# Autodesk Inventor assembly: EFOI-10
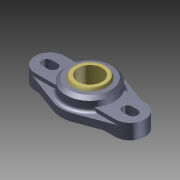
[picture p0: Inventor's stored thumbnail of the model, 180x180]
Saved by Autodesk Inventor 2011 (Build 150239000, 239)
## iProperties
Category: Plastic Bearings
Created: 2007-11-11
Part Number: EFOI-10
Catalog Web Link: http://www.igus.com/igcat/ig_cat1.asp?p=ig_27_2.gif
Description: igubal Flange Bearing
Vendor: igus
Document SubType Name: Assembly
Mass: 17.3933 g
Surface Area: 82.1485 cm^2
Volume: 15.021 cm^3
Density: 1.15793 g/cm^3
Project: FIRST
Title: igubal Flange Bearing
Author: Autodesk, Inc.
## Documents named in this file (3)
- R:\2012\Inventor\vkop\Plastic-Bearings\Plastic Bearings_igus_EFOI-10.iam
- R:\2012\Inventor\vkop\Plastic-Bearings\EFOI-10_Housing.ipt
- R:\2012\Inventor\vkop\Plastic-Bearings\EFOI-10_Spherical Bearing.ipt
## Components (2 placed, 2 different names)
1. EFOI-10_Housing:1 — Mate:1, Angle:1
2. EFOI-10_Spherical Bearing:1 — Mate:1, Angle:1
## Relationships (2: Mate 1, Angle 1)
- Mate:1: EFOI-10_Housing:1 ↔ EFOI-10_Spherical Bearing:1
- Angle:1 (0 deg): EFOI-10_Housing:1 ↔ EFOI-10_Spherical Bearing:1
